# Autodesk Inventor assembly: A2017_T3_07
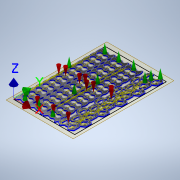
[picture p0: Inventor's stored thumbnail of the model, 180x180]
Saved by Autodesk Inventor 2022.3 (Build 263350000, 350)
## iProperties
Created: 2022-09-28
Part Number: A2017_T3_07
Document SubType Name: Assembly
Designer: Masato
Author: Masato
## Documents named in this file (4)
- C:\Users\Masato\Documents\Inventor\Inventor for CIT Brains\SUSTAINA-OP - cam\Cam\A2017_T3\A2017_T3_07.iam
- C:\Users\Masato\Documents\Inventor\Inventor for CIT Brains\SUSTAINA-OP - cam\Cam\DisposableBoard.ipt
- C:\Users\Masato\Documents\Inventor\Inventor for CIT Brains\SUSTAINA-OP - cam\LowerBody\Ankle\Ankle_front_frame.ipt
- C:\Users\Masato\Documents\Inventor\Inventor for CIT Brains\SUSTAINA-OP - cam\LowerBody\Leg_joint\Leg_joint_roll_frame.ipt
## Components (50 placed, 3 different names)
1. DisposableBoard:1 — フラッシュ:1, フラッシュ:2, フラッシュ:3, フラッシュ:4, フラッシュ:5, フラッシュ:6, フラッシュ:7
2. Ankle_front_frame:1 — メイト:1, フラッシュ:5, フラッシュ:6
3. Ankle_front_frame:2
4. Ankle_front_frame:3 — 正接:1, 正接:2, メイト:3
5. Ankle_front_frame:4
6. Ankle_front_frame:5
7. Ankle_front_frame:6
8. Ankle_front_frame:7
9. Ankle_front_frame:8
10. Ankle_front_frame:9
11. Ankle_front_frame:10
12. Ankle_front_frame:11
13. Ankle_front_frame:12
14. Ankle_front_frame:13
15. Ankle_front_frame:14
16. Ankle_front_frame:15
17. Ankle_front_frame:16
18. Ankle_front_frame:17
19. Ankle_front_frame:18
20. Ankle_front_frame:19
21. Ankle_front_frame:20
22. Ankle_front_frame:21
23. Ankle_front_frame:22
24. Ankle_front_frame:23
25. Ankle_front_frame:24
26. Ankle_front_frame:25
27. Ankle_front_frame:26
28. Ankle_front_frame:27
29. Ankle_front_frame:28
30. Ankle_front_frame:29
31. Ankle_front_frame:30
32. Ankle_front_frame:31
33. Ankle_front_frame:32
34. Ankle_front_frame:33
35. Ankle_front_frame:34
36. Ankle_front_frame:35
37. Ankle_front_frame:36
38. Ankle_front_frame:37
39. Ankle_front_frame:38
40. Ankle_front_frame:39
41. Leg_joint_roll_frame:1 — メイト:2, 正接:1, 正接:2, メイト:3, 正接:3
42. Leg_joint_roll_frame:2 — メイト:4, 正接:3, フラッシュ:7
43. Leg_joint_roll_frame:3
44. Leg_joint_roll_frame:4
45. Leg_joint_roll_frame:5
46. Leg_joint_roll_frame:6
47. Leg_joint_roll_frame:7
48. Leg_joint_roll_frame:8
49. Leg_joint_roll_frame:9
50. Leg_joint_roll_frame:10
## Component patterns: (39 elements, first: Ankle_front_frame:1), (5 elements, first: Leg_joint_roll_frame:1 + Leg_joint_roll_frame:2)
## Relationships (14: Flush 7, Mate 4, Tangent 3)
- フラッシュ:1 [Flush]: DisposableBoard:1
- フラッシュ:2 [Flush]: DisposableBoard:1
- フラッシュ:3 [Flush]: DisposableBoard:1
- フラッシュ:4 [Flush]: DisposableBoard:1
- メイト:1 [Mate]: Ankle_front_frame:1
- フラッシュ:5 [Flush] (-2 mm): DisposableBoard:1 ↔ Ankle_front_frame:1
- フラッシュ:6 [Flush] (2 mm): DisposableBoard:1 ↔ Ankle_front_frame:1
- メイト:2 [Mate]: Leg_joint_roll_frame:1
- 正接:1 [Tangent]: Ankle_front_frame:3 ↔ Leg_joint_roll_frame:1
- 正接:2 [Tangent]: Ankle_front_frame:3 ↔ Leg_joint_roll_frame:1
- メイト:3 [Mate] (2.1 mm): Ankle_front_frame:3 ↔ Leg_joint_roll_frame:1
- メイト:4 [Mate]: Leg_joint_roll_frame:2
- 正接:3 [Tangent] (2.1 mm): Leg_joint_roll_frame:1 ↔ Leg_joint_roll_frame:2
- フラッシュ:7 [Flush] (-2 mm): DisposableBoard:1 ↔ Leg_joint_roll_frame:2
